# Autodesk Inventor assembly: 42146-22
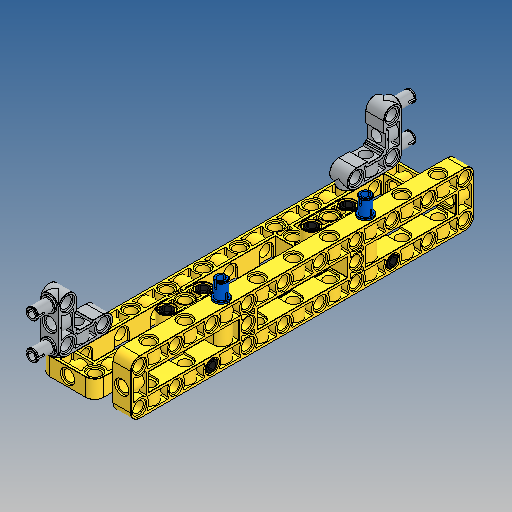
[picture p0: Inventor's stored thumbnail of the model, 512x512]
Saved by Autodesk Inventor 2025 (Build 290162010, 162A)
## iProperties
Created: 2024-11-23
Part Number: 42146-22
Material: Generisch
Document SubType Name: Assembly
Designer: hp.muther
Author: hp.muther
## Documents named in this file (7)
- D:\Inventor\Projekte\Muther\LEGO Technic\LEGO Technik - Raupenkran LR 13000 (42146)\42146-22.iam
- D:\Inventor\Projekte\Muther\LEGO Technic\LEGO Pieces\Rahmen, T-Stücke\67491-Yellow.ipt
- D:\Inventor\Projekte\Muther\LEGO Technic\LEGO Pieces\Pin's\2780-Black.ipt
- D:\Inventor\Projekte\Muther\LEGO Technic\LEGO Pieces\Pin's\6558-Blue.ipt
- D:\Inventor\Projekte\Muther\LEGO Technic\LEGO Pieces\Verbindungselemente\55615-LtBluishGray.ipt
- D:\Inventor\Projekte\Muther\LEGO Technic\LEGO Pieces\Rahmen, T-Stücke\60484-Yellow.ipt
- D:\Inventor\Projekte\Muther\LEGO Technic\LEGO Pieces\Lochbalken\32525-Yellow.ipt
## Components (17 placed, 6 different names)
1. 67491-Yellow:1 — Einfügen:1, Einfügen:2, Einfügen:5, Einfügen:6, Einfügen:7, Einfügen:8, Einfügen:11, Einfügen:12, Einfügen:13, Einfügen:14, Einfügen:15, Passend:4, Passend:5
2. 2780-Black:1 — Einfügen:1, Passend:1
3. 2780-Black:2 — Einfügen:2
4. 2780-Black:3 — Einfügen:3
5. 2780-Black:4 — Einfügen:4
6. 2780-Black:5 — Einfügen:5
7. 2780-Black:6 — Einfügen:6, Passend:3
8. 2780-Black:7 — Einfügen:7
9. 2780-Black:8 — Einfügen:8, Passend:2
10. 6558-Blue:1 — Einfügen:10, Passend:7
11. 6558-Blue:2 — Einfügen:9, Passend:6
12. 55615-LtBluishGray:1 — Einfügen:11, Passend:4
13. 55615-LtBluishGray:2 — Einfügen:12, Passend:5
14. 60484-Yellow:1 — Einfügen:13, Passend:2, Passend:7
15. 60484-Yellow:2 — Einfügen:14, Passend:3, Passend:6, Passend:8
16. 67491-Yellow:2 — Einfügen:9, Einfügen:10, Passend:8
17. 32525-Yellow:1 — Einfügen:3, Einfügen:4, Einfügen:15, Passend:1
## Relationships (23: Insert 15, Mate 8)
- Einfügen:1 [Insert]: 67491-Yellow:1 ↔ 2780-Black:1
- Einfügen:2 [Insert]: 67491-Yellow:1 ↔ 2780-Black:2
- Einfügen:3 [Insert]: 2780-Black:3 ↔ 32525-Yellow:1
- Einfügen:4 [Insert]: 2780-Black:4 ↔ 32525-Yellow:1
- Einfügen:5 [Insert]: 67491-Yellow:1 ↔ 2780-Black:5
- Einfügen:6 [Insert]: 67491-Yellow:1 ↔ 2780-Black:6
- Einfügen:7 [Insert]: 67491-Yellow:1 ↔ 2780-Black:7
- Einfügen:8 [Insert]: 67491-Yellow:1 ↔ 2780-Black:8
- Einfügen:9 [Insert]: 6558-Blue:2 ↔ 67491-Yellow:2
- Einfügen:10 [Insert]: 6558-Blue:1 ↔ 67491-Yellow:2
- Einfügen:11 [Insert]: 67491-Yellow:1 ↔ 55615-LtBluishGray:1
- Einfügen:12 [Insert]: 67491-Yellow:1 ↔ 55615-LtBluishGray:2
- Einfügen:13 [Insert]: 67491-Yellow:1 ↔ 60484-Yellow:1
- Einfügen:14 [Insert]: 67491-Yellow:1 ↔ 60484-Yellow:2
- Einfügen:15 [Insert]: 67491-Yellow:1 ↔ 32525-Yellow:1
- Passend:1 [Mate]: 2780-Black:1 ↔ 32525-Yellow:1
- Passend:2 [Mate]: 2780-Black:8 ↔ 60484-Yellow:1
- Passend:3 [Mate]: 2780-Black:6 ↔ 60484-Yellow:2
- Passend:4 [Mate]: 67491-Yellow:1 ↔ 55615-LtBluishGray:1
- Passend:5 [Mate]: 67491-Yellow:1 ↔ 55615-LtBluishGray:2
- Passend:6 [Mate]: 6558-Blue:2 ↔ 60484-Yellow:2
- Passend:7 [Mate]: 6558-Blue:1 ↔ 60484-Yellow:1
- Passend:8 [Mate]: 60484-Yellow:2 ↔ 67491-Yellow:2
